# Autodesk Inventor assembly: BagMotor-Assembly
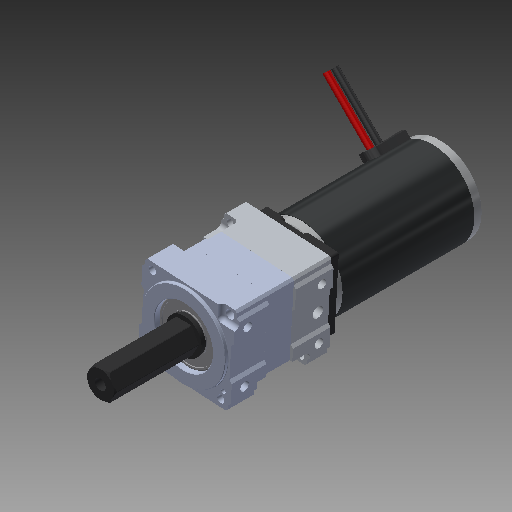
[picture p0: Inventor's stored thumbnail of the model, 512x512]
Saved by Autodesk Inventor 2017 (Build 210142000, 142)
## iProperties
Created: 2018-01-24
Part Number: BagMotor-Assembly
Document SubType Name: Assembly
Designer: Mentor
Author: Mentor
## Documents named in this file (9)
- E:\GrabCAD\Power Hawks CAD\Resources\VEXpro Resources\Motors\BagMotor-Assembly.iam
- E:\GrabCAD\Power Hawks CAD\Resources\VEXpro Resources\Motors\BagMotor-1111-2018.ipt
- E:\GrabCAD\Power Hawks CAD\Resources\VEXpro Resources\Gearboxes\Versaplanetary Gearbox with 775 Pro\217-2625-025 Rev1.ipt
- E:\GrabCAD\Power Hawks CAD\Resources\VEXpro Resources\Gearboxes\Versaplanetary Gearbox with 775 Pro\217-2816-001 Rev1.ipt
- E:\GrabCAD\Power Hawks CAD\Resources\VEXpro Resources\Gearboxes\Versaplanetary Gearbox with 775 Pro\217-2625-026 Rev1.ipt
- E:\GrabCAD\Power Hawks CAD\Resources\VEXpro Resources\Gearboxes\Versaplanetary Gearbox with 775 Pro\217-4649-006 Rev1_SSA0004-008BA.ipt
- E:\GrabCAD\Power Hawks CAD\Resources\VEXpro Resources\Gearboxes\Versaplanetary Gearbox with 775 Pro\217-2822-002 Rev4.ipt
- E:\GrabCAD\Power Hawks CAD\Resources\VEXpro Resources\Gearboxes\Versaplanetary Gearbox with 775 Pro\217-2742-001 Rev4.ipt
- E:\GrabCAD\Power Hawks CAD\Resources\VEXpro Resources\Gearboxes\Versaplanetary Gearbox with 775 Pro\217-2625-003 Rev1.ipt
## Components (8 placed, 8 different names)
1. BagMotor-1111-2018:1 — Mate:5, Mate:6, Mate:8
2. 217-2625-025 Rev1:1 — Mate:2, Flush:2, Mate:3, Mate:7, Flush:4
3. 217-2816-001 Rev1:1 — Mate:1, Mate:2, Flush:2, Flush:3, Mate:3, Mate:4, Mate:14
4. 217-2625-026 Rev1:1 — Mate:1, Flush:3, Mate:4, Mate:6, Mate:10, Mate:11, Mate:14
5. 217-4649-006 Rev1_SSA0004-008BA:1 — Mate:9
6. 217-2822-002 Rev4:1 — Mate:5, Mate:7, Flush:4, Mate:8, Mate:9
7. 217-2742-001 Rev4:1 — Mate:10, Mate:11, Mate:12, Mate:13
8. 217-2625-003 Rev1:1 — Mate:12, Mate:13
## Relationships (17: Mate 14, Flush 3)
- Mate:1: 217-2816-001 Rev1:1 ↔ 217-2625-026 Rev1:1
- Mate:2: 217-2625-025 Rev1:1 ↔ 217-2816-001 Rev1:1
- Flush:2: 217-2625-025 Rev1:1 ↔ 217-2816-001 Rev1:1
- Flush:3: 217-2816-001 Rev1:1 ↔ 217-2625-026 Rev1:1
- Mate:3: 217-2625-025 Rev1:1 ↔ 217-2816-001 Rev1:1
- Mate:4: 217-2816-001 Rev1:1 ↔ 217-2625-026 Rev1:1
- Mate:5: BagMotor-1111-2018:1 ↔ 217-2822-002 Rev4:1
- Mate:6: BagMotor-1111-2018:1 ↔ 217-2625-026 Rev1:1
- Mate:7: 217-2625-025 Rev1:1 ↔ 217-2822-002 Rev4:1
- Flush:4: 217-2625-025 Rev1:1 ↔ 217-2822-002 Rev4:1
- Mate:8: BagMotor-1111-2018:1 ↔ 217-2822-002 Rev4:1
- Mate:9: 217-4649-006 Rev1_SSA0004-008BA:1 ↔ 217-2822-002 Rev4:1
- Mate:10: 217-2625-026 Rev1:1 ↔ 217-2742-001 Rev4:1
- Mate:11: 217-2625-026 Rev1:1 ↔ 217-2742-001 Rev4:1
- Mate:12: 217-2742-001 Rev4:1 ↔ 217-2625-003 Rev1:1
- Mate:13: 217-2742-001 Rev4:1 ↔ 217-2625-003 Rev1:1
- Mate:14: 217-2816-001 Rev1:1 ↔ 217-2625-026 Rev1:1
